# Autodesk Inventor assembly: leftInsertbearing
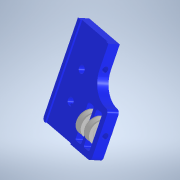
[picture p0: Inventor's stored thumbnail of the model, 180x180]
Saved by Autodesk Inventor 2020 (Build 240168000, 168)
## iProperties
Created: 2019-12-19
Part Number: leftInsertbearing
Document SubType Name: Assembly
Designer: xj82b
Author: xj82b
## Documents named in this file (3)
- C:\Users\xj82b\Documents\Inventor\5199\leftInsertbearing.iam
- C:\Users\xj82b\Documents\Inventor\5199\3x12x4mm-bearing.ipt
- C:\Users\xj82b\Documents\Inventor\5199\leftshortNEW.ipt
## Components (3 placed, 2 different names)
1. 3x12x4mm-bearing:1 — Mate:1, Mate:2
2. 3x12x4mm-bearing:2 — Mate:3, Mate:4
3. leftshortNEW:1 — Mate:1, Mate:2, Mate:3, Mate:4
## Relationships (4: Mate 4)
- Mate:1: 3x12x4mm-bearing:1 ↔ leftshortNEW:1
- Mate:2: 3x12x4mm-bearing:1 ↔ leftshortNEW:1
- Mate:3: 3x12x4mm-bearing:2 ↔ leftshortNEW:1
- Mate:4: 3x12x4mm-bearing:2 ↔ leftshortNEW:1
